# Autodesk Inventor assembly: HotBed_LM6021
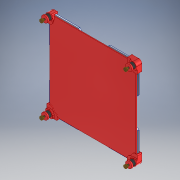
[picture p0: Inventor's stored thumbnail of the model, 180x180]
Saved by Autodesk Inventor 2020.3 (Build 243373000, 373)
## iProperties
Created: 2020-05-12
Part Number: HotBed_LM6021
Document SubType Name: Assembly
Designer: rah75
Author: rah75
## Documents named in this file (11)
- C:\Users\rah75\Documents\GitHub\LETU-Maker\CAD\Autodesk Inventor\Modules_6001-9999\HotBed\Assemblies\HotBed_LM6021.iam
- C:\Users\rah75\Documents\GitHub\LETU-Maker\CAD\Autodesk Inventor\Modules_6001-9999\HotBed\Printed_Parts\HotBed_Corner_Bracket_LN6016.ipt
- C:\Users\rah75\Documents\GitHub\LETU-Maker\CAD\Autodesk Inventor\Modules_6001-9999\HotBed\Fabricated_Parts\HotBed_Glass_200x200_LM6017.ipt
- C:\Users\rah75\Documents\GitHub\LETU-Maker\CAD\Autodesk Inventor\Modules_6001-9999\HotBed\Fabricated_Parts\HotBed_Plate_LM6018.ipt
- C:\Users\rah75\Documents\GitHub\LETU-Maker\CAD\Autodesk Inventor\Modules_6001-9999\HotBed\Printed_Parts\HotBed_Corner_Bracket_Clipped_LN6019.ipt
- C:\Users\rah75\Documents\GitHub\LETU-Maker\CAD\Autodesk Inventor\Modules_6001-9999\HotBed\Fabricated_Parts\HotBed_PCB_LM6020.ipt
- C:\Users\rah75\Documents\GitHub\LETU-Maker\CAD\Autodesk Inventor\Stock_Components_1001-2999\Fasteners\Washers_Spacers\Rubber_Grommet_5mmIDx13mmODx10mm_LM1046.ipt
- C:\Users\rah75\Documents\GitHub\LETU-Maker\CAD\Autodesk Inventor\Stock_Components_1001-2999\Fasteners\Nuts\hex_nut_m3_LM1019.ipt
- C:\Users\rah75\Documents\GitHub\LETU-Maker\CAD\Autodesk Inventor\Stock_Components_1001-2999\Fasteners\Nuts\thumb_nut_LM1047.ipt
- C:\Users\rah75\Documents\GitHub\LETU-Maker\CAD\Autodesk Inventor\Modules_6001-9999\HotBed\Printed_Parts\Rubber_Gromment_Cap_LM6015.ipt
- C:\Users\rah75\Documents\GitHub\LETU-Maker\CAD\Autodesk Inventor\Stock_Components_1001-2999\Fasteners\Screws\SHCS_m3x30_LM1012.ipt
## Components (27 placed, 10 different names)
1. HotBed_Glass_200x200_LM6017:1 — Mate:1, Mate:2, Angle:1
2. HotBed_Plate_LM6018:1 — Mate:1, Mate:2, Insert:1, Angle:1, Angle:2, Insert:2, Insert:3, Insert:4, Insert:5
3. HotBed_Corner_Bracket_LN6016:2 — Insert:3, Flush:1, Insert:6, Insert:11
4. HotBed_Corner_Bracket_LN6016:3 — Insert:2, Flush:1, Insert:7, Insert:10
5. HotBed_Corner_Bracket_LN6016:4 — Insert:1, Angle:2, Flush:2, Mate:3, Insert:8, Insert:13
6. HotBed_Corner_Bracket_Clipped_LN6019:1 — Insert:4, Flush:2, Insert:9, Insert:12
7. HotBed_PCB_LM6020:1 — Insert:5, Mate:3
8. Rubber_Grommet_5mmIDx13mmODx10mm_LM1046:1 — Insert:13, Insert:21
9. Rubber_Grommet_5mmIDx13mmODx10mm_LM1046:2 — Insert:12, Insert:20
10. Rubber_Grommet_5mmIDx13mmODx10mm_LM1046:3 — Insert:11, Insert:19
11. Rubber_Grommet_5mmIDx13mmODx10mm_LM1046:4 — Insert:10, Insert:18
12. hex_nut_m3_LM1019:1 — Insert:9
13. hex_nut_m3_LM1019:2 — Insert:8
14. hex_nut_m3_LM1019:3 — Insert:7
15. hex_nut_m3_LM1019:4 — Insert:6
16. SHCS_m3x30_LM1012:1
17. SHCS_m3x30_LM1012:2
18. SHCS_m3x30_LM1012:3
19. SHCS_m3x30_LM1012:4
20. thumb_nut_LM1047:1 — Insert:25
21. thumb_nut_LM1047:2 — Insert:23
22. thumb_nut_LM1047:3 — Insert:22
23. thumb_nut_LM1047:4 — Insert:24
24. Rubber_Gromment_Cap_LM6015:1 — Insert:20, Insert:24
25. Rubber_Gromment_Cap_LM6015:2 — Insert:18, Insert:22
26. Rubber_Gromment_Cap_LM6015:3 — Insert:19, Insert:23
27. Rubber_Gromment_Cap_LM6015:4 — Insert:21, Insert:25
## Relationships (32: Insert 25, Mate 3, Angle 2, Flush 2)
- Mate:1: HotBed_Glass_200x200_LM6017:1 ↔ HotBed_Plate_LM6018:1
- Mate:2: HotBed_Glass_200x200_LM6017:1 ↔ HotBed_Plate_LM6018:1
- Insert:1: HotBed_Plate_LM6018:1 ↔ HotBed_Corner_Bracket_LN6016:4
- Angle:1 (0 deg): HotBed_Glass_200x200_LM6017:1 ↔ HotBed_Plate_LM6018:1
- Angle:2 (0 deg): HotBed_Plate_LM6018:1 ↔ HotBed_Corner_Bracket_LN6016:4
- Insert:2: HotBed_Plate_LM6018:1 ↔ HotBed_Corner_Bracket_LN6016:3
- Insert:3: HotBed_Plate_LM6018:1 ↔ HotBed_Corner_Bracket_LN6016:2
- Flush:1: HotBed_Corner_Bracket_LN6016:2 ↔ HotBed_Corner_Bracket_LN6016:3
- Insert:4: HotBed_Plate_LM6018:1 ↔ HotBed_Corner_Bracket_Clipped_LN6019:1
- Flush:2: HotBed_Corner_Bracket_LN6016:4 ↔ HotBed_Corner_Bracket_Clipped_LN6019:1
- Insert:5: HotBed_Plate_LM6018:1 ↔ HotBed_PCB_LM6020:1
- Mate:3: HotBed_Corner_Bracket_LN6016:4 ↔ HotBed_PCB_LM6020:1
- Insert:6: HotBed_Corner_Bracket_LN6016:2 ↔ hex_nut_m3_LM1019:4
- Insert:7: HotBed_Corner_Bracket_LN6016:3 ↔ hex_nut_m3_LM1019:3
- Insert:8: HotBed_Corner_Bracket_LN6016:4 ↔ hex_nut_m3_LM1019:2
- Insert:9: HotBed_Corner_Bracket_Clipped_LN6019:1 ↔ hex_nut_m3_LM1019:1
- Insert:10: HotBed_Corner_Bracket_LN6016:3 ↔ Rubber_Grommet_5mmIDx13mmODx10mm_LM1046:4
- Insert:11: HotBed_Corner_Bracket_LN6016:2 ↔ Rubber_Grommet_5mmIDx13mmODx10mm_LM1046:3
- Insert:12: HotBed_Corner_Bracket_Clipped_LN6019:1 ↔ Rubber_Grommet_5mmIDx13mmODx10mm_LM1046:2
- Insert:13: HotBed_Corner_Bracket_LN6016:4 ↔ Rubber_Grommet_5mmIDx13mmODx10mm_LM1046:1
- [Insert]: HotBed_Plate_LM6018:1 ↔ SHCS_m3x30_LM1012:1
- [Insert]: HotBed_Plate_LM6018:1 ↔ SHCS_m3x30_LM1012:2
- [Insert]: HotBed_Plate_LM6018:1 ↔ SHCS_m3x30_LM1012:3
- [Insert]: HotBed_Plate_LM6018:1 ↔ SHCS_m3x30_LM1012:4
- Insert:18: Rubber_Grommet_5mmIDx13mmODx10mm_LM1046:4 ↔ Rubber_Gromment_Cap_LM6015:2
- Insert:19: Rubber_Grommet_5mmIDx13mmODx10mm_LM1046:3 ↔ Rubber_Gromment_Cap_LM6015:3
- Insert:20: Rubber_Grommet_5mmIDx13mmODx10mm_LM1046:2 ↔ Rubber_Gromment_Cap_LM6015:1
- Insert:21: Rubber_Grommet_5mmIDx13mmODx10mm_LM1046:1 ↔ Rubber_Gromment_Cap_LM6015:4
- Insert:22 (3.175 mm): thumb_nut_LM1047:3 ↔ Rubber_Gromment_Cap_LM6015:2
- Insert:23 (3.175 mm): thumb_nut_LM1047:2 ↔ Rubber_Gromment_Cap_LM6015:3
- Insert:24 (3.175 mm): thumb_nut_LM1047:4 ↔ Rubber_Gromment_Cap_LM6015:1
- Insert:25 (3.175 mm): thumb_nut_LM1047:1 ↔ Rubber_Gromment_Cap_LM6015:4
